# Autodesk Inventor assembly: L3 Gearbox Assembly_MIR
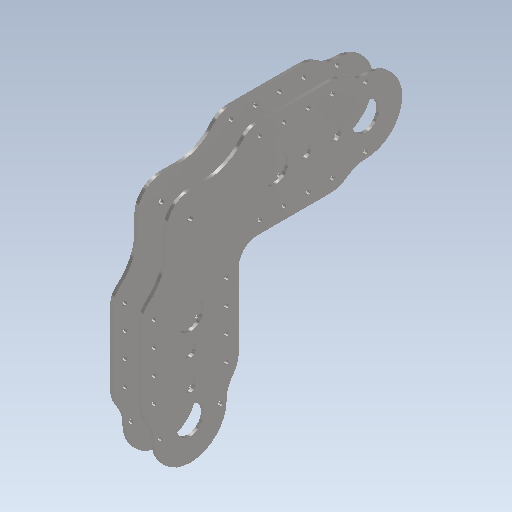
[picture p0: Inventor's stored thumbnail of the model, 512x512]
Saved by Autodesk Inventor 2023 (Build 270158000, 158)
## iProperties
Created: 2023-02-14
Part Number: L3 Gearbox Assembly_MIR
Document SubType Name: Assembly
Designer: Dave
Mass: 1965.41 g
Surface Area: 3646.76 cm^2
Volume: 537.619 cm^3
Density: 3.65577 g/cm^3
Author: Dave
## Documents named in this file (3)
- C:\Users\Dave\Documents\GitHub\BehrendURCMechanical\CAD\Chassis V3\L3 Gearbox Assembly_MIR.iam
- C:\Users\Dave\Documents\GitHub\BehrendURCMechanical\CAD\Chassis V3\L3Plate_MIR.ipt
- C:\Users\Dave\Documents\GitHub\BehrendURCMechanical\CAD\Chassis\GearBox\CH-1-01-0.25IDSmoothBoreBearing_MIR1.ipt
## Components (3 placed, 2 different names)
1. L3Plate_MIR:1 — Angle:1, Flush:2
2. L3Plate_MIR:2 — Insert:9, Flush:2
3. CH-1-01-0.25IDSmoothBoreBearing_MIR1:1 — Insert:9
## Relationships (3: Angle 1, Insert 1, Flush 1)
- Angle:1 (0 deg): L3Plate_MIR:1
- Insert:9: L3Plate_MIR:2 ↔ CH-1-01-0.25IDSmoothBoreBearing_MIR1:1
- Flush:2: L3Plate_MIR:1 ↔ L3Plate_MIR:2
